# Autodesk Inventor assembly: Plataforma 4dof
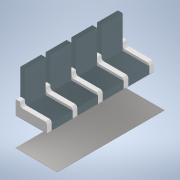
[picture p0: Inventor's stored thumbnail of the model, 180x180]
Saved by Autodesk Inventor 2021 (Build 250183000, 183)
## iProperties
Created: 2021-03-18
Part Number: Plataforma 4dof
Document SubType Name: Assembly
Designer: andre
Author: andre
## Documents named in this file (5)
- C:\Users\andre\Documents\GitHub\Dis.-Mecatronico-E6\Inventor\Plataforma 4dof.iam
- C:\Users\andre\Documents\GitHub\Dis.-Mecatronico-E6\Inventor\placa inferior.ipt
- C:\Users\andre\Documents\GitHub\Dis.-Mecatronico-E6\Inventor\placa superior.ipt
- C:\Users\andre\Documents\GitHub\Dis.-Mecatronico-E6\Inventor\silla.ipt
- C:\Users\andre\Documents\GitHub\Dis.-Mecatronico-E6\Inventor\bracera.ipt
## Components (11 placed, 4 different names)
1. placa inferior:1 — Flush:1
2. placa superior:1 — Flush:2, Flush:3, Flush:4, Flush:5
3. silla:1 — Flush:4, Flush:5, Rigid:1, Flush:6, Flush:7, Rigid:4
4. silla:2 — Rigid:1, Rigid:2, Rigid:7
5. silla:3 — Rigid:2, Rigid:3
6. silla:4 — Rigid:3, Rigid:5, Rigid:6
7. bracera:1 — Flush:6, Flush:7
8. bracera:2 — Rigid:4
9. bracera:3 — Rigid:5
10. bracera:4 — Rigid:6
11. bracera:5 — Rigid:7
## Relationships (14: Flush 7, WeldJoint 7)
- Flush:1 (600 mm): placa inferior:1
- Flush:2: placa superior:1
- Flush:3: placa superior:1
- Flush:4: placa superior:1 ↔ silla:1
- Flush:5: placa superior:1 ↔ silla:1
- Rigid:1 [WeldJoint] (100 mm): silla:1 ↔ silla:2
- Rigid:2 [WeldJoint] (100 mm): silla:2 ↔ silla:3
- Rigid:3 [WeldJoint] (100 mm): silla:3 ↔ silla:4
- Flush:6: silla:1 ↔ bracera:1
- Flush:7: silla:1 ↔ bracera:1
- Rigid:4 [WeldJoint]: silla:1 ↔ bracera:2
- Rigid:5 [WeldJoint]: silla:4 ↔ bracera:3
- Rigid:6 [WeldJoint]: silla:4 ↔ bracera:4
- Rigid:7 [WeldJoint]: silla:2 ↔ bracera:5
